# Autodesk Inventor assembly: RGBCube
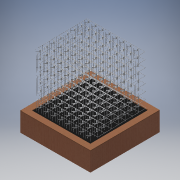
[picture p0: Inventor's stored thumbnail of the model, 180x180]
Saved by Autodesk Inventor 2019.3 (Build 233278000, 278)
## iProperties
Created: 2019-01-14
Part Number: RGBCube
Material: Generisch
Document SubType Name: Assembly
Designer: Jonas
Author: Jonas
## Documents named in this file (5)
- C:\Users\Jonas\Desktop\RGBCube\RGBCubev2\CAD\RGBCube.iam
- C:\Users\Jonas\Desktop\RGBCube\RGBCubev2\CAD\Socket\CompleteSocket.iam
- C:\Users\Jonas\Desktop\RGBCube\RGBCubev2\CAD\Led\LedCube.iam
- C:\Users\Jonas\Desktop\RGBCube\RGBCubev2\CAD\PCBs\ShiftRegisters.iam
- C:\Users\Jonas\Desktop\RGBCube\RGBCubev2\CAD\PCBs\ShiftRegisters.ipt
## Components (5 placed, 3 different names)
1. CompleteSocket:1 [sub-assembly] — Passend:1, Passend:2, Passend:3, Passend:4, Passend:5, Passend:6, Passend:7, Passend:8, Passend:9, Passend:10, Passend:11
2. LedCube:1 [sub-assembly] — Passend:3, Passend:4, Passend:5
3. ShiftRegisters:1 [sub-assembly] — Passend:6, Passend:7
4. ShiftRegisters:2 — Passend:8, Passend:9
5. ShiftRegisters:3 — Passend:10, Passend:11
## Relationships (11: Mate 11)
- Passend:1 [Mate]: CompleteSocket:1
- Passend:2 [Mate]: CompleteSocket:1
- Passend:3 [Mate] (-7 mm): CompleteSocket:1 ↔ LedCube:1
- Passend:4 [Mate] (15.5 mm): CompleteSocket:1 ↔ LedCube:1
- Passend:5 [Mate] (-15 mm): CompleteSocket:1 ↔ LedCube:1
- Passend:6 [Mate]: CompleteSocket:1 ↔ ShiftRegisters:1
- Passend:7 [Mate]: CompleteSocket:1 ↔ ShiftRegisters:1
- Passend:8 [Mate]: CompleteSocket:1 ↔ ShiftRegisters:2
- Passend:9 [Mate]: CompleteSocket:1 ↔ ShiftRegisters:2
- Passend:10 [Mate]: CompleteSocket:1 ↔ ShiftRegisters:3
- Passend:11 [Mate]: CompleteSocket:1 ↔ ShiftRegisters:3
